# Autodesk Inventor assembly: LazySusan
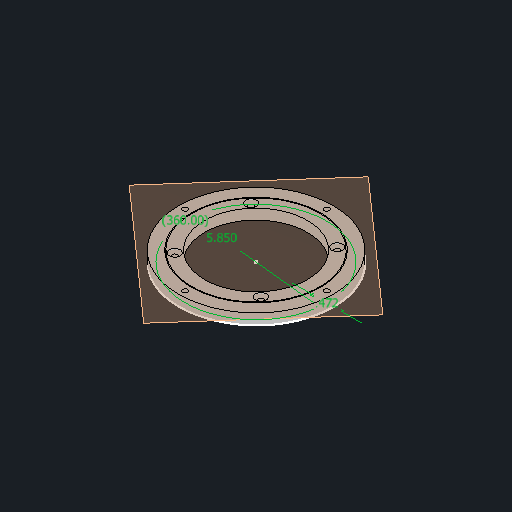
[picture p0: Inventor's stored thumbnail of the model, 512x512]
Saved by Autodesk Inventor 2024 (Build 280153000, 153)
## iProperties
Created: 2023-10-21
Part Number: LazySusan
Document SubType Name: Assembly
Designer: range
Author: range
## Documents named in this file (3)
- C:\Users\range\CodingProjects\C-AAM\CAD\V1\Parts\LazySusan.iam
- C:\Users\range\CodingProjects\C-AAM\CAD\V1\OR.ipt
- C:\Users\range\CodingProjects\C-AAM\CAD\V1\IR.ipt
## Components (2 placed, 2 different names)
1. OR:1 — Flush:1, Flush:2, Mate:1
2. IR:1 — Flush:1, Flush:2, Mate:1
## Relationships (3: Flush 2, Mate 1)
- Flush:1: OR:1 ↔ IR:1
- Flush:2: OR:1 ↔ IR:1
- Mate:1: OR:1 ↔ IR:1
